# Autodesk Inventor assembly: 組合3
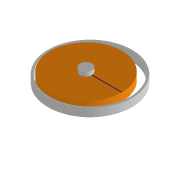
[picture p0: Inventor's stored thumbnail of the model, 180x180]
Saved by Autodesk Inventor 2022 (Build 260153000, 153)
## iProperties
Created: 2023-05-26
Part Number: 組合3
Document SubType Name: Assembly
Designer: JOU
Author: JOU
## Documents named in this file (4)
- C:\Users\JOU\Desktop\git\Special-project\接觸解析器練習資料夾\接觸解析器練習資料夾\Cycloidal Gear\組合3.iam
- C:\Users\JOU\Desktop\git\Special-project\接觸解析器練習資料夾\接觸解析器練習資料夾\Cycloidal Gear\t1.ipt
- C:\Users\JOU\Desktop\git\Special-project\接觸解析器練習資料夾\接觸解析器練習資料夾\Cycloidal Gear\t2.ipt
- C:\Users\JOU\Desktop\git\Special-project\接觸解析器練習資料夾\接觸解析器練習資料夾\Cycloidal Gear\t3.ipt
## Components (3 placed, 3 different names)
1. t1:1 — 齊平:1, 貼合:1, 角度:1
2. t2:1 — 齊平:1, 齊平:2, 貼合:2, 角度:1, 旋轉:1
3. t3:1 — 貼合:1, 齊平:2, 貼合:2, 旋轉:1
## Relationships (6: Flush 2, Mate 2, Angle 1, RelateRotation 1)
- 齊平:1 [Flush]: t1:1 ↔ t2:1
- 貼合:1 [Mate]: t1:1 ↔ t3:1
- 齊平:2 [Flush]: t2:1 ↔ t3:1
- 貼合:2 [Mate]: t2:1 ↔ t3:1
- 角度:1 [Angle] (0 deg): t1:1 ↔ t2:1
- 旋轉:1 [RelateRotation] (9 ul): t2:1 ↔ t3:1
